# Autodesk Inventor assembly: Robot
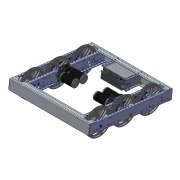
[picture p0: Inventor's stored thumbnail of the model, 180x180]
Saved by Autodesk Inventor 2016 (Build 200138000, 138)
## iProperties
Created: 2016-01-27
Part Number: Robot
Document SubType Name: Assembly
Designer: PrashantBIA
Author: PrashantBIA
## Documents named in this file (9)
- C:\Users\PrashantBIA\Desktop\Robotics\Robot Assembly\Robot.iam
- C:\Users\PrashantBIA\Desktop\Robotics\Robot Assembly\Drive Train\AM14U3+Square+REV1-1.iam
- C:\Users\PrashantBIA\Desktop\Robotics\Robot Assembly\Electronic Parts\CIM Motor.ipt
- C:\Users\PrashantBIA\Desktop\Robotics\Robot Assembly\1x1\22in.ipt
- C:\Users\PrashantBIA\Desktop\Robotics\Robot Assembly\Electronic Parts\Electrical Board Assembly.iam
- C:\Users\PrashantBIA\Desktop\Robotics\Robot Assembly\Electronic Parts\am-2939+BatteryHolder.ipt
- C:\Users\PrashantBIA\Desktop\Robotics\Robot Assembly\Electronic Parts\ELEC_Battery_NP18-12B.ipt
- C:\Users\PrashantBIA\Desktop\Robotics\Robot Assembly\Special Assemblies\8inWheel.iam
- C:\Users\PrashantBIA\Desktop\Robotics\Robot Assembly\Special Assemblies\Middle8inWheel.iam
## Components (16 placed, 8 different names)
1. CIM Motor:4 — Insert:2
2. CIM Motor:3 — Insert:1
3. CIM Motor:2 — Insert:3
4. CIM Motor:1 — Insert:4
5. AM14U3+Square+REV1-1:1 [sub-assembly] — Insert:1, Insert:2, Flush:1, Mate:15, Mate:16, Flush:2, Mate:19, Mate:20, Mate:21, Mate:24, Mate:25, Mate:26, Mate:27, Mate:28, Mate:30, Mate:31, Mate:32, Mate:33, Mate:35, Mate:36, Mate:38, Insert:3, Insert:4, Mate:39, Mate:40, Mate:41
6. 22in:1 — Flush:1, Mate:15, Mate:17, Flush:4
7. 22in:2 — Mate:16, Flush:2, Mate:17, Flush:3, Mate:18
8. Electrical Board Assembly:1 [sub-assembly] — Flush:3, Mate:18, Flush:4
9. am-2939+BatteryHolder:1 — Mate:19, Mate:20, Mate:21, Mate:22, Mate:23
10. ELEC_Battery_NP18-12B:1 — Mate:22, Mate:23, Mate:24
11. Middle8inWheel:2 [sub-assembly] — Mate:36, Mate:39
12. Middle8inWheel:1 [sub-assembly] — Mate:35, Mate:38
13. 8inWheel:4 [sub-assembly] — Mate:28, Mate:41
14. 8inWheel:3 [sub-assembly] — Mate:32, Mate:33, Mate:40
15. 8inWheel:2 [sub-assembly] — Mate:30, Mate:31
16. 8inWheel:1 [sub-assembly] — Mate:25, Mate:26, Mate:27
## Relationships (32: Mate 24, Insert 4, Flush 4)
- Insert:1: CIM Motor:3 ↔ AM14U3+Square+REV1-1:1
- Insert:2: CIM Motor:4 ↔ AM14U3+Square+REV1-1:1
- Flush:1: AM14U3+Square+REV1-1:1 ↔ 22in:1
- Mate:15: AM14U3+Square+REV1-1:1 ↔ 22in:1
- Mate:16: AM14U3+Square+REV1-1:1 ↔ 22in:2
- Flush:2: AM14U3+Square+REV1-1:1 ↔ 22in:2
- Mate:17 (304.8 mm): 22in:1 ↔ 22in:2
- Flush:3: 22in:2 ↔ Electrical Board Assembly:1
- Mate:18: 22in:2 ↔ Electrical Board Assembly:1
- Flush:4 (-76.2 mm): 22in:1 ↔ Electrical Board Assembly:1
- Mate:19: AM14U3+Square+REV1-1:1 ↔ am-2939+BatteryHolder:1
- Mate:20: AM14U3+Square+REV1-1:1 ↔ am-2939+BatteryHolder:1
- Mate:21: AM14U3+Square+REV1-1:1 ↔ am-2939+BatteryHolder:1
- Mate:22: am-2939+BatteryHolder:1 ↔ ELEC_Battery_NP18-12B:1
- Mate:23: am-2939+BatteryHolder:1 ↔ ELEC_Battery_NP18-12B:1
- Mate:24: AM14U3+Square+REV1-1:1 ↔ ELEC_Battery_NP18-12B:1
- Mate:25: AM14U3+Square+REV1-1:1 ↔ 8inWheel:1
- Mate:26: AM14U3+Square+REV1-1:1 ↔ 8inWheel:1
- Mate:27: AM14U3+Square+REV1-1:1 ↔ 8inWheel:1
- Mate:28: AM14U3+Square+REV1-1:1 ↔ 8inWheel:4
- Mate:30: AM14U3+Square+REV1-1:1 ↔ 8inWheel:2
- Mate:31: AM14U3+Square+REV1-1:1 ↔ 8inWheel:2
- Mate:32: AM14U3+Square+REV1-1:1 ↔ 8inWheel:3
- Mate:33: AM14U3+Square+REV1-1:1 ↔ 8inWheel:3
- Mate:35: AM14U3+Square+REV1-1:1 ↔ Middle8inWheel:1
- Mate:36: AM14U3+Square+REV1-1:1 ↔ Middle8inWheel:2
- Mate:38: AM14U3+Square+REV1-1:1 ↔ Middle8inWheel:1
- Insert:3: CIM Motor:2 ↔ AM14U3+Square+REV1-1:1
- Insert:4: CIM Motor:1 ↔ AM14U3+Square+REV1-1:1
- Mate:39: AM14U3+Square+REV1-1:1 ↔ Middle8inWheel:2
- Mate:40: AM14U3+Square+REV1-1:1 ↔ 8inWheel:3
- Mate:41: AM14U3+Square+REV1-1:1 ↔ 8inWheel:4
